# Autodesk Inventor assembly: Rail_AssemblyV2_0
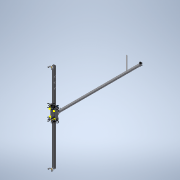
[picture p0: Inventor's stored thumbnail of the model, 180x180]
Saved by Autodesk Inventor 2021 (Build 250183000, 183)
## iProperties
Created: 2021-01-25
Part Number: Rail_AssemblyV2_0
Document SubType Name: Assembly
Designer: Jorian Brusind
Mass: 3786.54 g
Surface Area: 19508.5 cm^2
Volume: 2323.9 cm^3
Density: 1.62939 g/cm^3
Author: Jorian Brusind
## Documents named in this file (25)
- C:\Users\Jorian Bruslind\Documents\GitHub\PersonalProjects\HyperRail\Inventor Files\Rail_AssemblyV2_0.iam
- C:\Users\Jorian Bruslind\Documents\GitHub\PersonalProjects\Inventor Projects\Useful models\NEMA_Steppers\NEMA23\23HS8430B.ipt
- C:\Users\Jorian Bruslind\Documents\GitHub\PersonalProjects\HyperRail\Inventor Files\2804S_NEMA2115_1Gearbox.ipt
- C:\Users\Jorian Bruslind\Documents\GitHub\PersonalProjects\HyperRail\PCB Files\Integrated Stepper Motor Driver\ExportSTEP\Main.iam
- C:\Users\Jorian Bruslind\Documents\GitHub\PersonalProjects\HyperRail\Inventor Files\NEMA23_Shroud.ipt
- C:\Users\Jorian Bruslind\Documents\GitHub\PersonalProjects\Inventor Projects\Useful models\8020_Sets\IPT_20_Series\IPT_20_Series\20-4040_2m.ipt
- C:\Users\Jorian Bruslind\Documents\GitHub\PersonalProjects\HyperRail\Inventor Files\98952A059_ALUM MALE-FEM THRDED HEX STANDOFF.ipt
- C:\Users\Jorian Bruslind\Documents\GitHub\PersonalProjects\HyperRail\Inventor Files\95783A039_NYLON 6-6 MALE-FEM THRDED HEX STANDOFF.ipt
- C:\Users\Jorian Bruslind\Documents\GitHub\PersonalProjects\HyperRail\Inventor Files\Integrated_Stepper_NEMA23_Mount.ipt
- C:\Users\Jorian Bruslind\Documents\GitHub\PersonalProjects\Inventor Projects\Useful models\8020_Sets\IPT_40_Series\Extra_40_Series\HFS5-4060-4000\HFS5-4060-2125.ipt
- C:\Users\Jorian Bruslind\Documents\GitHub\PersonalProjects\Inventor Projects\Useful models\8020_Sets\AIS2018\20-2568_d.iam
- C:\Users\Jorian Bruslind\Documents\GitHub\PersonalProjects\HyperRail\Inventor Files\5mm_bore_10mm_width_idlepulley.ipt
- C:\Users\Jorian Bruslind\Documents\GitHub\PersonalProjects\HyperRail\Inventor Files\Idler_Spacer.ipt
- C:\Users\Jorian Bruslind\Documents\GitHub\PersonalProjects\HyperRail\Inventor Files\Tape_Belt_Layer.ipt
- C:\Users\Jorian Bruslind\Documents\GitHub\PersonalProjects\HyperRail\Inventor Files\SDP_sdpsi_a_6a55m028df0912\SDP_sdpsi_a_6a55m028df0912.ipt
- C:\Users\Jorian Bruslind\Documents\GitHub\PersonalProjects\HyperRail\Inventor Files\SDP_sdpsi_a_6r25mc250\SDP_sdpsi_a_6r25mc1000.ipt
- C:\Users\Jorian Bruslind\Documents\GitHub\PersonalProjects\Inventor Projects\Useful models\8020_Sets\IPT_20_Series\Extra_20_Series\8020_14056m\14056_m.ipt
- C:\Users\Jorian Bruslind\Documents\GitHub\PersonalProjects\HyperRail\Inventor Files\Cable_Guide_Holder.ipt
- C:\Users\Jorian Bruslind\Documents\GitHub\PersonalProjects\HyperRail\Inventor Files\Carriage_Assembly.iam
- C:\Users\Jorian Bruslind\Documents\GitHub\PersonalProjects\HyperRail\Inventor Files\NEMA23_StepperonlineMount.ipt
- C:\Users\Jorian Bruslind\Documents\GitHub\PersonalProjects\HyperRail\Inventor Files\59145_Sensor.ipt
- C:\Users\Jorian Bruslind\Documents\GitHub\PersonalProjects\HyperRail\Inventor Files\RightAngle_SideBracket.ipt
- C:\Users\Jorian Bruslind\Documents\GitHub\PersonalProjects\HyperRail\Inventor Files\Bottom_Foot_Standoff.ipt
- C:\Users\Jorian Bruslind\Documents\GitHub\PersonalProjects\HyperRail\Inventor Files\SpacerBlock_25mm.ipt
- C:\Users\Jorian Bruslind\Documents\GitHub\PersonalProjects\HyperRail\Inventor Files\McMaster Files\Leveling Feet\62805K49_Heavy Duty Leveling Mount.ipt
## Components (53 placed, 24 different names)
1. 23HS8430B:1 — Mate:127, Angle:3, Mate:158, Mate:177, Mate:179, Mate:180, Mate:181, Mate:182, Mate:183, Mate:184, Mate:185, Mate:264, Mate:265, Mate:295, Angle:5, Angle:6
2. 2804S_NEMA2115_1Gearbox:1 — Mate:127, Angle:3, Mate:158, Flush:86, Mate:336, Flush:126, Mate:370, Mate:371
3. Main:1 [sub-assembly] — Mate:291, Mate:292, Mate:293
4. 20-4040_2m:2 — Flush:123, Mate:322, Mate:323, Mate:326, Mate:327, Mate:330, Mate:331, Mate:345, Mate:346, Mate:354, Flush:143, Mate:374, Flush:156, Mate:375, Flush:158, Mate:377, Mate:378, Flush:160, Flush:161, Flush:163
5. NEMA23_Shroud:1 — Mate:264, Mate:265, Flush:86, Angle:7
6. 98952A059_ALUM MALE-FEM THRDED HEX STANDOFF:1 — Mate:180, Mate:181, Mate:186, Mate:191
7. 98952A059_ALUM MALE-FEM THRDED HEX STANDOFF:2 — Mate:184, Mate:185, Mate:189, Mate:192
8. 98952A059_ALUM MALE-FEM THRDED HEX STANDOFF:3 — Mate:177, Mate:179, Mate:187, Mate:190
9. 98952A059_ALUM MALE-FEM THRDED HEX STANDOFF:4 — Mate:182, Mate:183, Mate:188, Mate:193
10. 95783A039_NYLON 6-6 MALE-FEM THRDED HEX STANDOFF:1 — Mate:188, Mate:193
11. 95783A039_NYLON 6-6 MALE-FEM THRDED HEX STANDOFF:2 — Mate:186, Mate:191, Mate:369
12. 95783A039_NYLON 6-6 MALE-FEM THRDED HEX STANDOFF:3 — Mate:187, Mate:190
13. 95783A039_NYLON 6-6 MALE-FEM THRDED HEX STANDOFF:4 — Mate:189, Mate:192
14. HFS5-4060-2125:1 — Mate:277, Mate:278, Mate:279, Mate:280, Mate:332, Mate:333, Mate:344, Flush:132, Flush:133, Mate:347, Mate:348, Mate:349, Flush:141, Flush:142, Mate:353, Mate:366, Flush:167, Mate:393, Flush:168, Flush:169, Mate:409, Mate:410, Flush:176, Flush:177, Flush:178
15. Integrated_Stepper_NEMA23_Mount:1 — Mate:291, Mate:292, Mate:293, Mate:295, Mate:360, Mate:361, Mate:362, Mate:363, Mate:364, Mate:369, Angle:5, Angle:6
16. 20-2568_d:1 [sub-assembly] — Flush:123, Mate:322, Mate:323
17. 5mm_bore_10mm_width_idlepulley:1 — Mate:324, Mate:325, Angle:4
18. Idler_Spacer:1 — Mate:324, Mate:325, Mate:326, Mate:327
19. 5mm_bore_10mm_width_idlepulley:2 — Mate:328, Mate:329, Angle:4
20. Idler_Spacer:2 — Mate:328, Mate:329, Mate:330, Mate:331
21. Tape_Belt_Layer:1 — Mate:332, Mate:333
22. SDP_sdpsi_a_6a55m028df0912:1 — Mate:336, Flush:126
23. SDP_sdpsi_a_6r25mc1000:1 — Flush:130, Mate:343, Flush:131, Mate:344, Flush:132, Flush:133
24. SDP_sdpsi_a_6r25mc1000:2 — Flush:130, Mate:343, Flush:131, Flush:148, Flush:149
25. 14056_m:1 — Mate:346, Flush:144, Flush:146
26. 14056_m:3 — Mate:345, Flush:145, Flush:146, Mate:355
27. Cable_Guide_Holder:1 — Mate:348, Flush:136, Mate:350, Mate:351, Flush:140
28. Cable_Guide_Holder:2 — Mate:347, Mate:350, Flush:140, Flush:142
29. Cable_Guide_Holder:3 — Mate:349, Flush:136, Mate:351, Flush:141
30. Carriage_Assembly:1 [sub-assembly] — Mate:353, Mate:354, Flush:143, Flush:144, Flush:145, Mate:355, Mate:366, Mate:372, Flush:153, Mate:373, Flush:154, Flush:155, Flush:157, Flush:159, Mate:376
31. SDP_sdpsi_a_6r25mc1000:3 — Flush:148, Flush:149
32. 98952A059_ALUM MALE-FEM THRDED HEX STANDOFF:5 — Mate:360, Flush:151, Flush:152
33. 98952A059_ALUM MALE-FEM THRDED HEX STANDOFF:6 — Mate:361, Flush:152
34. 98952A059_ALUM MALE-FEM THRDED HEX STANDOFF:7 — Mate:362, Mate:364, Flush:150, Flush:151
35. 98952A059_ALUM MALE-FEM THRDED HEX STANDOFF:8 — Mate:363, Flush:150
36. NEMA23_StepperonlineMount:1 — Mate:370, Mate:371, Angle:7, Mate:372, Flush:153
37. 59145_Sensor:1 — Mate:373, Flush:154, Flush:155
38. RightAngle_SideBracket:1 — Mate:375, Flush:158, Flush:159
39. RightAngle_SideBracket:2 — Mate:374, Flush:156, Flush:157, Mate:376
40. RightAngle_SideBracket:3 — Mate:378, Flush:160, Flush:162, Flush:163
41. RightAngle_SideBracket:4 — Mate:377, Flush:161, Flush:162
42. Bottom_Foot_Standoff:2 — Flush:167, Mate:394, Mate:395, Flush:170, Mate:396, Mate:397, Mate:398
43. SpacerBlock_25mm:1 — Mate:393, Flush:168, Flush:169, Mate:394, Mate:395, Flush:170
44. 62805K49_Heavy Duty Leveling Mount:1 — Mate:396, Flush:171, Mate:398
45. 62805K49_Heavy Duty Leveling Mount:2 — Mate:397, Flush:171
46. Bottom_Foot_Standoff:3
47. SpacerBlock_25mm:2 — Mate:410, Flush:178, Mate:411
48. 62805K49_Heavy Duty Leveling Mount:3
49. 62805K49_Heavy Duty Leveling Mount:4
50. Bottom_Foot_Standoff:4
51. SpacerBlock_25mm:3 — Mate:409, Flush:176, Flush:177, Mate:411
52. 62805K49_Heavy Duty Leveling Mount:5
53. 62805K49_Heavy Duty Leveling Mount:6
## Relationships (136: Mate 88, Flush 43, Angle 5)
- Mate:127: 23HS8430B:1 ↔ 2804S_NEMA2115_1Gearbox:1
- Angle:3 (0 deg): 23HS8430B:1 ↔ 2804S_NEMA2115_1Gearbox:1
- Mate:158: 23HS8430B:1 ↔ 2804S_NEMA2115_1Gearbox:1
- Mate:177: 23HS8430B:1 ↔ 98952A059_ALUM MALE-FEM THRDED HEX STANDOFF:3
- Mate:179: 23HS8430B:1 ↔ 98952A059_ALUM MALE-FEM THRDED HEX STANDOFF:3
- Mate:180: 23HS8430B:1 ↔ 98952A059_ALUM MALE-FEM THRDED HEX STANDOFF:1
- Mate:181: 23HS8430B:1 ↔ 98952A059_ALUM MALE-FEM THRDED HEX STANDOFF:1
- Mate:182: 23HS8430B:1 ↔ 98952A059_ALUM MALE-FEM THRDED HEX STANDOFF:4
- Mate:183: 23HS8430B:1 ↔ 98952A059_ALUM MALE-FEM THRDED HEX STANDOFF:4
- Mate:184: 23HS8430B:1 ↔ 98952A059_ALUM MALE-FEM THRDED HEX STANDOFF:2
- Mate:185: 23HS8430B:1 ↔ 98952A059_ALUM MALE-FEM THRDED HEX STANDOFF:2
- Mate:186: 98952A059_ALUM MALE-FEM THRDED HEX STANDOFF:1 ↔ 95783A039_NYLON 6-6 MALE-FEM THRDED HEX STANDOFF:2
- Mate:187: 98952A059_ALUM MALE-FEM THRDED HEX STANDOFF:3 ↔ 95783A039_NYLON 6-6 MALE-FEM THRDED HEX STANDOFF:3
- Mate:188: 98952A059_ALUM MALE-FEM THRDED HEX STANDOFF:4 ↔ 95783A039_NYLON 6-6 MALE-FEM THRDED HEX STANDOFF:1
- Mate:189: 98952A059_ALUM MALE-FEM THRDED HEX STANDOFF:2 ↔ 95783A039_NYLON 6-6 MALE-FEM THRDED HEX STANDOFF:4
- Mate:190: 98952A059_ALUM MALE-FEM THRDED HEX STANDOFF:3 ↔ 95783A039_NYLON 6-6 MALE-FEM THRDED HEX STANDOFF:3
- Mate:191: 98952A059_ALUM MALE-FEM THRDED HEX STANDOFF:1 ↔ 95783A039_NYLON 6-6 MALE-FEM THRDED HEX STANDOFF:2
- Mate:192: 98952A059_ALUM MALE-FEM THRDED HEX STANDOFF:2 ↔ 95783A039_NYLON 6-6 MALE-FEM THRDED HEX STANDOFF:4
- Mate:193: 98952A059_ALUM MALE-FEM THRDED HEX STANDOFF:4 ↔ 95783A039_NYLON 6-6 MALE-FEM THRDED HEX STANDOFF:1
- Mate:264 (1 mm): 23HS8430B:1 ↔ NEMA23_Shroud:1
- Mate:265 (1 mm): 23HS8430B:1 ↔ NEMA23_Shroud:1
- Flush:86: 2804S_NEMA2115_1Gearbox:1 ↔ NEMA23_Shroud:1
- Mate:277: HFS5-4060-2125:1
- Mate:278: HFS5-4060-2125:1
- Mate:279: HFS5-4060-2125:1
- Mate:280: HFS5-4060-2125:1
- Mate:291: Main:1 ↔ Integrated_Stepper_NEMA23_Mount:1
- Mate:292: Main:1 ↔ Integrated_Stepper_NEMA23_Mount:1
- Mate:293: Main:1 ↔ Integrated_Stepper_NEMA23_Mount:1
- Mate:295: 23HS8430B:1 ↔ Integrated_Stepper_NEMA23_Mount:1
- Flush:123: 20-4040_2m:2 ↔ 20-2568_d:1
- Mate:322 (-2 mm): 20-4040_2m:2 ↔ 20-2568_d:1
- Mate:323: 20-4040_2m:2 ↔ 20-2568_d:1
- Mate:324: 5mm_bore_10mm_width_idlepulley:1 ↔ Idler_Spacer:1
- Mate:325: 5mm_bore_10mm_width_idlepulley:1 ↔ Idler_Spacer:1
- Mate:326: 20-4040_2m:2 ↔ Idler_Spacer:1
- Mate:327 (2.5 mm): 20-4040_2m:2 ↔ Idler_Spacer:1
- Mate:328: 5mm_bore_10mm_width_idlepulley:2 ↔ Idler_Spacer:2
- Mate:329: 5mm_bore_10mm_width_idlepulley:2 ↔ Idler_Spacer:2
- Mate:330: 20-4040_2m:2 ↔ Idler_Spacer:2
- Mate:331 (2.5 mm): 20-4040_2m:2 ↔ Idler_Spacer:2
- Angle:4 (0 deg): 5mm_bore_10mm_width_idlepulley:1 ↔ 5mm_bore_10mm_width_idlepulley:2
- Mate:332: HFS5-4060-2125:1 ↔ Tape_Belt_Layer:1
- Mate:333 (1 mm): HFS5-4060-2125:1 ↔ Tape_Belt_Layer:1
- Mate:336: 2804S_NEMA2115_1Gearbox:1 ↔ SDP_sdpsi_a_6a55m028df0912:1
- Flush:126: 2804S_NEMA2115_1Gearbox:1 ↔ SDP_sdpsi_a_6a55m028df0912:1
- Flush:130: SDP_sdpsi_a_6r25mc1000:1 ↔ SDP_sdpsi_a_6r25mc1000:2
- Mate:343: SDP_sdpsi_a_6r25mc1000:1 ↔ SDP_sdpsi_a_6r25mc1000:2
- Flush:131: SDP_sdpsi_a_6r25mc1000:1 ↔ SDP_sdpsi_a_6r25mc1000:2
- Mate:344 (1 mm): HFS5-4060-2125:1 ↔ SDP_sdpsi_a_6r25mc1000:1
- Flush:132: HFS5-4060-2125:1 ↔ SDP_sdpsi_a_6r25mc1000:1
- Flush:133: HFS5-4060-2125:1 ↔ SDP_sdpsi_a_6r25mc1000:1
- Mate:345: 20-4040_2m:2 ↔ 14056_m:3
- Mate:346: 20-4040_2m:2 ↔ 14056_m:1
- Mate:347: HFS5-4060-2125:1 ↔ Cable_Guide_Holder:2
- Mate:348: HFS5-4060-2125:1 ↔ Cable_Guide_Holder:1
- Mate:349: HFS5-4060-2125:1 ↔ Cable_Guide_Holder:3
- Flush:136: Cable_Guide_Holder:1 ↔ Cable_Guide_Holder:3
- Mate:350 (100 mm): Cable_Guide_Holder:1 ↔ Cable_Guide_Holder:2
- Mate:351 (100 mm): Cable_Guide_Holder:1 ↔ Cable_Guide_Holder:3
- Flush:140: Cable_Guide_Holder:1 ↔ Cable_Guide_Holder:2
- Flush:141 (-20 mm): HFS5-4060-2125:1 ↔ Cable_Guide_Holder:3
- Flush:142 (200 mm): HFS5-4060-2125:1 ↔ Cable_Guide_Holder:2
- Mate:353 (6 mm): HFS5-4060-2125:1 ↔ Carriage_Assembly:1
- Mate:354: 20-4040_2m:2 ↔ Carriage_Assembly:1
- Flush:143: 20-4040_2m:2 ↔ Carriage_Assembly:1
- Flush:144: 14056_m:1 ↔ Carriage_Assembly:1
- Flush:145: 14056_m:3 ↔ Carriage_Assembly:1
- Flush:146: 14056_m:1 ↔ 14056_m:3
- Mate:355: 14056_m:3 ↔ Carriage_Assembly:1
- Flush:148 (2.5 mm): SDP_sdpsi_a_6r25mc1000:2 ↔ SDP_sdpsi_a_6r25mc1000:3
- Flush:149: SDP_sdpsi_a_6r25mc1000:2 ↔ SDP_sdpsi_a_6r25mc1000:3
- Mate:360: Integrated_Stepper_NEMA23_Mount:1 ↔ 98952A059_ALUM MALE-FEM THRDED HEX STANDOFF:5
- Mate:361: Integrated_Stepper_NEMA23_Mount:1 ↔ 98952A059_ALUM MALE-FEM THRDED HEX STANDOFF:6
- Mate:362: Integrated_Stepper_NEMA23_Mount:1 ↔ 98952A059_ALUM MALE-FEM THRDED HEX STANDOFF:7
- Mate:363: Integrated_Stepper_NEMA23_Mount:1 ↔ 98952A059_ALUM MALE-FEM THRDED HEX STANDOFF:8
- Mate:364: Integrated_Stepper_NEMA23_Mount:1 ↔ 98952A059_ALUM MALE-FEM THRDED HEX STANDOFF:7
- Flush:150: 98952A059_ALUM MALE-FEM THRDED HEX STANDOFF:7 ↔ 98952A059_ALUM MALE-FEM THRDED HEX STANDOFF:8
- Flush:151: 98952A059_ALUM MALE-FEM THRDED HEX STANDOFF:5 ↔ 98952A059_ALUM MALE-FEM THRDED HEX STANDOFF:7
- Flush:152: 98952A059_ALUM MALE-FEM THRDED HEX STANDOFF:5 ↔ 98952A059_ALUM MALE-FEM THRDED HEX STANDOFF:6
- Mate:366 (22.5 mm): HFS5-4060-2125:1 ↔ Carriage_Assembly:1
- Mate:369: 95783A039_NYLON 6-6 MALE-FEM THRDED HEX STANDOFF:2 ↔ Integrated_Stepper_NEMA23_Mount:1
- Angle:5 (0 deg): 23HS8430B:1 ↔ Integrated_Stepper_NEMA23_Mount:1
- Angle:6 (0 deg): 23HS8430B:1 ↔ Integrated_Stepper_NEMA23_Mount:1
- Mate:370: 2804S_NEMA2115_1Gearbox:1 ↔ NEMA23_StepperonlineMount:1
- Mate:371: 2804S_NEMA2115_1Gearbox:1 ↔ NEMA23_StepperonlineMount:1
- Angle:7 (0 deg): NEMA23_Shroud:1 ↔ NEMA23_StepperonlineMount:1
- Mate:372: Carriage_Assembly:1 ↔ NEMA23_StepperonlineMount:1
- Flush:153 (-11.25 mm): Carriage_Assembly:1 ↔ NEMA23_StepperonlineMount:1
- Mate:373: Carriage_Assembly:1 ↔ 59145_Sensor:1
- Flush:154 (5 mm): Carriage_Assembly:1 ↔ 59145_Sensor:1
- Flush:155: Carriage_Assembly:1 ↔ 59145_Sensor:1
- Mate:374: 20-4040_2m:2 ↔ RightAngle_SideBracket:2
- Flush:156: 20-4040_2m:2 ↔ RightAngle_SideBracket:2
- Flush:157: Carriage_Assembly:1 ↔ RightAngle_SideBracket:2
- Mate:375: 20-4040_2m:2 ↔ RightAngle_SideBracket:1
- Flush:158: 20-4040_2m:2 ↔ RightAngle_SideBracket:1
- Flush:159: Carriage_Assembly:1 ↔ RightAngle_SideBracket:1
- Mate:376: Carriage_Assembly:1 ↔ RightAngle_SideBracket:2
- Mate:377: 20-4040_2m:2 ↔ RightAngle_SideBracket:4
- Mate:378: 20-4040_2m:2 ↔ RightAngle_SideBracket:3
- Flush:160: 20-4040_2m:2 ↔ RightAngle_SideBracket:3
- Flush:161: 20-4040_2m:2 ↔ RightAngle_SideBracket:4
- Flush:162: RightAngle_SideBracket:3 ↔ RightAngle_SideBracket:4
- Flush:163 (-20 mm): 20-4040_2m:2 ↔ RightAngle_SideBracket:3
- Flush:167: HFS5-4060-2125:1 ↔ Bottom_Foot_Standoff:2
- Mate:393: HFS5-4060-2125:1 ↔ SpacerBlock_25mm:1
- Flush:168: HFS5-4060-2125:1 ↔ SpacerBlock_25mm:1
- Flush:169 (20 mm): HFS5-4060-2125:1 ↔ SpacerBlock_25mm:1
- Mate:394: Bottom_Foot_Standoff:2 ↔ SpacerBlock_25mm:1
- Mate:395: Bottom_Foot_Standoff:2 ↔ SpacerBlock_25mm:1
- Flush:170: Bottom_Foot_Standoff:2 ↔ SpacerBlock_25mm:1
- Mate:396: Bottom_Foot_Standoff:2 ↔ 62805K49_Heavy Duty Leveling Mount:1
- Mate:397: Bottom_Foot_Standoff:2 ↔ 62805K49_Heavy Duty Leveling Mount:2
- Flush:171: 62805K49_Heavy Duty Leveling Mount:1 ↔ 62805K49_Heavy Duty Leveling Mount:2
- Mate:398 (20 mm): Bottom_Foot_Standoff:2 ↔ 62805K49_Heavy Duty Leveling Mount:1
- [Mate]: Bottom_Foot_Standoff:3 ↔ SpacerBlock_25mm:2
- [Mate]: Bottom_Foot_Standoff:3 ↔ SpacerBlock_25mm:2
- [Flush]: Bottom_Foot_Standoff:3 ↔ SpacerBlock_25mm:2
- [Mate]: Bottom_Foot_Standoff:3 ↔ 62805K49_Heavy Duty Leveling Mount:3
- [Mate]: Bottom_Foot_Standoff:3 ↔ 62805K49_Heavy Duty Leveling Mount:4
- [Flush]: 62805K49_Heavy Duty Leveling Mount:3 ↔ 62805K49_Heavy Duty Leveling Mount:4
- [Mate] (20 mm): Bottom_Foot_Standoff:3 ↔ 62805K49_Heavy Duty Leveling Mount:3
- [Mate]: Bottom_Foot_Standoff:4 ↔ SpacerBlock_25mm:3
- [Mate]: Bottom_Foot_Standoff:4 ↔ SpacerBlock_25mm:3
- [Flush]: Bottom_Foot_Standoff:4 ↔ SpacerBlock_25mm:3
- [Mate]: Bottom_Foot_Standoff:4 ↔ 62805K49_Heavy Duty Leveling Mount:5
- [Mate]: Bottom_Foot_Standoff:4 ↔ 62805K49_Heavy Duty Leveling Mount:6
- [Flush]: 62805K49_Heavy Duty Leveling Mount:5 ↔ 62805K49_Heavy Duty Leveling Mount:6
- [Mate] (20 mm): Bottom_Foot_Standoff:4 ↔ 62805K49_Heavy Duty Leveling Mount:5
- Mate:409: HFS5-4060-2125:1 ↔ SpacerBlock_25mm:3
- Mate:410: HFS5-4060-2125:1 ↔ SpacerBlock_25mm:2
- Flush:176: HFS5-4060-2125:1 ↔ SpacerBlock_25mm:3
- Flush:177 (20 mm): HFS5-4060-2125:1 ↔ SpacerBlock_25mm:3
- Flush:178 (20 mm): HFS5-4060-2125:1 ↔ SpacerBlock_25mm:2
- Mate:411 (1000 mm): SpacerBlock_25mm:2 ↔ SpacerBlock_25mm:3
## Named parameters: d763_d759 = 0 mm, d764_d760 = 0 mm, d765_d761 = 0 mm, d766_d762 = 20 mm, d767_d752 = 0 mm, d768_d753 = 0 mm, d769_d754 = 0 mm, d770_d759 = 0 mm, d771_d760 = 0 mm, d772_d761 = 0 mm, d773_d762 = 20 mm, d774_d752 = 0 mm, d775_d753 = 0 mm, d776_d754 = 0 mm
